# Autodesk Inventor assembly: Assembly of platform without top
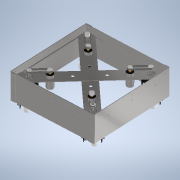
[picture p0: Inventor's stored thumbnail of the model, 180x180]
Saved by Autodesk Inventor 2020 (Build 240168000, 168)
## iProperties
Created: 2022-07-06
Part Number: Assembly of platform without top
Document SubType Name: Assembly
Designer: karimi2
Author: karimi2
## Documents named in this file (3)
- C:\Users\karimi2\Documents\PROJECT\src\Assembly of platform without top.iam
- C:\Users\karimi2\Documents\PROJECT\src\Wheels on Chassis Assembly.iam
- C:\Users\karimi2\Documents\PROJECT\src\Platform Sides Assembly.iam
## Components (2 placed, 2 different names)
1. Wheels on Chassis Assembly:1 [sub-assembly] — Mate:1, Mate:2, Mate:3, Mate:4, Mate:5, Mate:6
2. Platform Sides Assembly:1 [sub-assembly] — Mate:1, Mate:2, Mate:3, Mate:4, Mate:5, Mate:6
## Relationships (6: Mate 6)
- Mate:1: Wheels on Chassis Assembly:1 ↔ Platform Sides Assembly:1
- Mate:2: Wheels on Chassis Assembly:1 ↔ Platform Sides Assembly:1
- Mate:3: Wheels on Chassis Assembly:1 ↔ Platform Sides Assembly:1
- Mate:4: Wheels on Chassis Assembly:1 ↔ Platform Sides Assembly:1
- Mate:5: Wheels on Chassis Assembly:1 ↔ Platform Sides Assembly:1
- Mate:6: Wheels on Chassis Assembly:1 ↔ Platform Sides Assembly:1
